# Autodesk Inventor assembly: Nanoscopy-on-a-cheap_v0
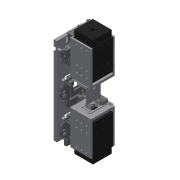
[picture p0: Inventor's stored thumbnail of the model, 180x180]
Saved by Autodesk Inventor 2019 (Build 230136000, 136)
## iProperties
Created: 2019-04-21
Part Number: Nanoscopy-on-a-cheap_v0
Document SubType Name: Assembly
Designer: diederichbenedict
Author: diederichbenedict
## Documents named in this file (4)
- C:\Users\diederichbenedict\Dropbox\Dokumente\Promotion\PROJECTS\STORMoChip\INVENTOR\Nanoscopy-on-a-cheap\Nanoscopy-on-a-cheap_v0.iam
- C:\Users\diederichbenedict\Dropbox\Dokumente\Promotion\PROJECTS\STORMoChip\INVENTOR\Nanoscopy-on-a-cheap\Assembly_Lasergroup_wPickup.iam
- C:\Users\diederichbenedict\Dropbox\Dokumente\Promotion\PROJECTS\STORMoChip\INVENTOR\Nanoscopy-on-a-cheap\Assembly_Chipgroup.iam
- C:\Users\diederichbenedict\Dropbox\Dokumente\Promotion\PROJECTS\STORMoChip\INVENTOR\Nanoscopy-on-a-cheap\10_Baseplate_XY.ipt
## Components (4 placed, 3 different names)
1. Assembly_Lasergroup_wPickup:1 [sub-assembly] — Mate:1, Flush:1, Flush:5
2. Assembly_Lasergroup_wPickup:2 [sub-assembly] — Mate:1, Flush:1, Flush:6
3. Assembly_Chipgroup:1 [sub-assembly]
4. 10_Baseplate_XY:1 — Flush:5, Flush:6
## Relationships (9: Flush 6, Mate 3)
- Mate:1: Assembly_Lasergroup_wPickup:1 ↔ Assembly_Lasergroup_wPickup:2
- Flush:1: Assembly_Lasergroup_wPickup:1 ↔ Assembly_Lasergroup_wPickup:2
- [Flush] (16 mm): Assembly_Lasergroup_wPickup:2 ↔ Assembly_Chipgroup:1
- [Flush]: Assembly_Lasergroup_wPickup:1 ↔ Assembly_Chipgroup:1
- [Mate] (3 mm): Assembly_Lasergroup_wPickup:1 ↔ Assembly_Chipgroup:1
- [Mate] (3 mm): Assembly_Lasergroup_wPickup:2 ↔ Assembly_Chipgroup:1
- [Flush]: Assembly_Lasergroup_wPickup:1 ↔ Assembly_Chipgroup:1
- Flush:5: Assembly_Lasergroup_wPickup:1 ↔ 10_Baseplate_XY:1
- Flush:6: Assembly_Lasergroup_wPickup:2 ↔ 10_Baseplate_XY:1
